# Autodesk Inventor assembly: Assy_CORE_board
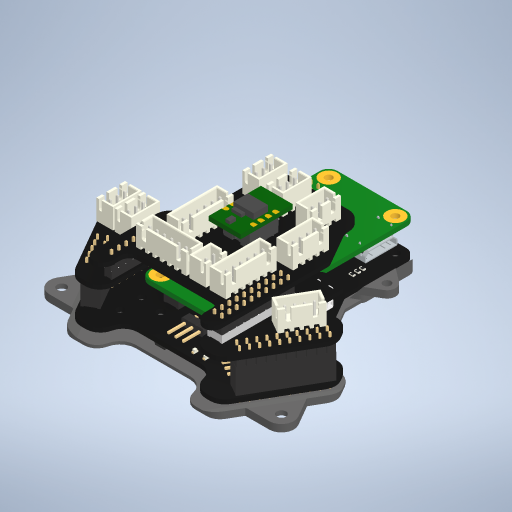
[picture p0: Inventor's stored thumbnail of the model, 512x512]
Saved by Autodesk Inventor 2024.1 (Build 281209000, 209)
## iProperties
Created: 2025-05-06
Part Number: Assy_CORE_board
Document SubType Name: Assembly
Designer: hibik
Author: hibik
## Documents named in this file (3)
- C:\Users\hibik\Documents\Robomech\RESCUE\ORCA\hard\flame_base\Assy_CORE_board.iam
- C:\Users\hibik\Documents\Robomech\RESCUE\ORCA\hard\board\CORE_model\CORE.iam
- C:\Users\hibik\Documents\Robomech\RESCUE\ORCA\hard\flame_base\CORE_board_setter.ipt
## Components (2 placed, 2 different names)
1. CORE_board_setter:1 — 挿入:1
2. CORE:1 [sub-assembly] — 挿入:1, 角度:1
## Relationships (2: Insert 1, Angle 1)
- 挿入:1 [Insert]: CORE_board_setter:1 ↔ CORE:1
- 角度:1 [Angle] (0 deg): CORE:1
